# Autodesk Inventor assembly: Dribbler
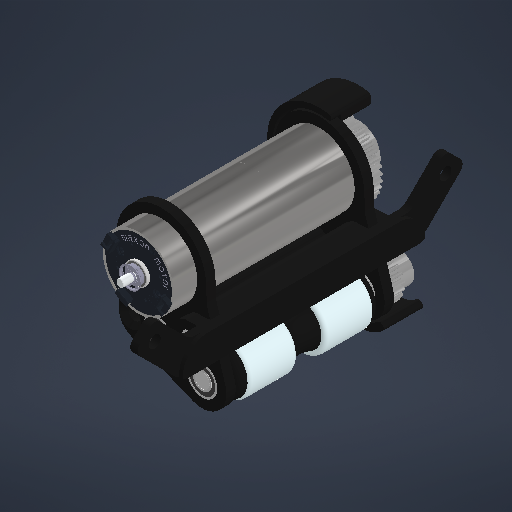
[picture p0: Inventor's stored thumbnail of the model, 512x512]
Saved by Autodesk Inventor 2026.1 (Build 301233020, 233B)
## iProperties
Created: 2025-12-15
Part Number: Dribbler
Document SubType Name: Assembly
Designer: Bahaa
Author: Bahaa
## Documents named in this file (16)
- C:\Users\Bahaa\Nextcloud2\CAD\25-26\Dribbler\Dribbler.iam
- C:\Users\Bahaa\Nextcloud2\CAD\25-26\Dribbler\Dribbler Bracket.ipt
- C:\Users\Bahaa\Nextcloud2\CAD\25-26\Parts\Miniatur Kugellager MR 84 2RS 4x8x3 mm.ipt
- C:\Users\Bahaa\Nextcloud2\CAD\25-26\Motoren\Maxon DCX 19mm 13W\DCX 19mm 13W.iam
- C:\Users\Bahaa\Nextcloud2\CAD\25-26\Dribbler\21102000.ipt
- C:\Users\Bahaa\Nextcloud2\CAD\25-26\Dribbler\21103000.ipt
- C:\Users\Bahaa\Nextcloud2\CAD\25-26\Dribbler\21104000.ipt
- C:\Users\Bahaa\Nextcloud2\CAD\25-26\Dribbler\Dribbler Bracket B.ipt
- C:\Users\Bahaa\Nextcloud2\CAD\25-26\Dribbler\M4 Dribbler Shaft.ipt
- C:\Users\Bahaa\Nextcloud2\CAD\25-26\Dribbler\Dribbler Roller.ipt
- C:\Users\Bahaa\Nextcloud2\CAD\25-26\Dribbler\Dribbler Roller Seperator.ipt
- C:\Users\Bahaa\Nextcloud2\CAD\25-26\Dribbler\Dribbler Support.ipt
- C:\Users\Bahaa\Nextcloud2\CAD\25-26\Dribbler\Dribbler Cover.ipt
- C:\Users\Bahaa\Nextcloud2\CAD\25-26\Dribbler\Dribber Shaft Hull.ipt
- C:\Users\Bahaa\Nextcloud2\CAD\25-26\Dribbler\Dribbler Mount.ipt
- C:\Users\Bahaa\Nextcloud2\CAD\25-26\Dribbler\Pivot M3 Shaft.ipt
## Components (20 placed, 15 different names)
1. Dribbler Bracket:1 — Mate:1, Mate:2, Flush:1, Flush:2, Mate:3, Mate:4, Mate:5, Mate:6, Mate:8, Mate:10, Mate:15, Mate:26, Mate:27, Mate:31, Mate:34, Transitional:1
2. Miniatur Kugellager MR 84 2RS 4x8x3 mm:1 — Mate:1, Flush:2, Mate:9
3. Miniatur Kugellager MR 84 2RS 4x8x3 mm:2 — Mate:2, Flush:1, Mate:11, Mate:36
4. DCX 19mm 13W:1 [sub-assembly] — Mate:3, Mate:4, Mate:5, Mate:7, Mate:12, Flush:5
5. 21102000:1 — Mate:10, Mate:11, Mate:17, Flush:7
6. 21103000:1 — Mate:8, Mate:9, Mate:16, Flush:6
7. 21104000:1 — Mate:6, Mate:7
8. Dribbler Bracket B:1 — Mate:12, Flush:3, Mate:13, Flush:4, Mate:14, Mate:15, Flush:5, Mate:24, Mate:25, Mate:30
9. Miniatur Kugellager MR 84 2RS 4x8x3 mm:3 — Flush:3, Mate:13
10. Miniatur Kugellager MR 84 2RS 4x8x3 mm:4 — Flush:4, Mate:14
11. M4 Dribbler Shaft:1 — Mate:16, Flush:6, Mate:29
12. M4 Dribbler Shaft:2 — Mate:17, Flush:7, Mate:19, Mate:21, Mate:23
13. Dribbler Roller:1 — Mate:19, Mate:38
14. Dribbler Roller:2 — Mate:21, Mate:37
15. Dribbler Roller Seperator:1 — Mate:23, Mate:36, Mate:37, Mate:38
16. Dribbler Support:1 — Mate:24, Mate:25
17. Dribbler Cover:1 — Mate:26, Mate:27, Mate:31
18. Dribber Shaft Hull:1 — Mate:29, Mate:30
19. Dribbler Mount:1 — Mate:32, Mate:33, Flush:8, Mate:34, Mate:35, Flush:9
20. Pivot M3 Shaft:1 — Mate:35, Flush:9, Transitional:1
## Relationships (44: Mate 34, Flush 9, Transitional 1)
- Mate:1: Dribbler Bracket:1 ↔ Miniatur Kugellager MR 84 2RS 4x8x3 mm:1
- Mate:2: Dribbler Bracket:1 ↔ Miniatur Kugellager MR 84 2RS 4x8x3 mm:2
- Flush:1: Dribbler Bracket:1 ↔ Miniatur Kugellager MR 84 2RS 4x8x3 mm:2
- Flush:2: Dribbler Bracket:1 ↔ Miniatur Kugellager MR 84 2RS 4x8x3 mm:1
- Mate:3: Dribbler Bracket:1 ↔ DCX 19mm 13W:1
- Mate:4: Dribbler Bracket:1 ↔ DCX 19mm 13W:1
- Mate:5: Dribbler Bracket:1 ↔ DCX 19mm 13W:1
- Mate:6: Dribbler Bracket:1 ↔ 21104000:1
- Mate:7: DCX 19mm 13W:1 ↔ 21104000:1
- Mate:8: Dribbler Bracket:1 ↔ 21103000:1
- Mate:9: Miniatur Kugellager MR 84 2RS 4x8x3 mm:1 ↔ 21103000:1
- Mate:10: Dribbler Bracket:1 ↔ 21102000:1
- Mate:11: Miniatur Kugellager MR 84 2RS 4x8x3 mm:2 ↔ 21102000:1
- Mate:12: DCX 19mm 13W:1 ↔ Dribbler Bracket B:1
- Flush:3: Dribbler Bracket B:1 ↔ Miniatur Kugellager MR 84 2RS 4x8x3 mm:3
- Mate:13: Dribbler Bracket B:1 ↔ Miniatur Kugellager MR 84 2RS 4x8x3 mm:3
- Flush:4: Dribbler Bracket B:1 ↔ Miniatur Kugellager MR 84 2RS 4x8x3 mm:4
- Mate:14: Dribbler Bracket B:1 ↔ Miniatur Kugellager MR 84 2RS 4x8x3 mm:4
- Mate:15: Dribbler Bracket:1 ↔ Dribbler Bracket B:1
- Flush:5 (-6 mm): DCX 19mm 13W:1 ↔ Dribbler Bracket B:1
- Mate:16: 21103000:1 ↔ M4 Dribbler Shaft:1
- Flush:6: 21103000:1 ↔ M4 Dribbler Shaft:1
- Mate:17: 21102000:1 ↔ M4 Dribbler Shaft:2
- Flush:7: 21102000:1 ↔ M4 Dribbler Shaft:2
- Mate:19: M4 Dribbler Shaft:2 ↔ Dribbler Roller:1
- Mate:21: M4 Dribbler Shaft:2 ↔ Dribbler Roller:2
- Mate:23: M4 Dribbler Shaft:2 ↔ Dribbler Roller Seperator:1
- Mate:24: Dribbler Bracket B:1 ↔ Dribbler Support:1
- Mate:25: Dribbler Bracket B:1 ↔ Dribbler Support:1
- Mate:26: Dribbler Bracket:1 ↔ Dribbler Cover:1
- Mate:27: Dribbler Bracket:1 ↔ Dribbler Cover:1
- Mate:29: M4 Dribbler Shaft:1 ↔ Dribber Shaft Hull:1
- Mate:30: Dribbler Bracket B:1 ↔ Dribber Shaft Hull:1
- Mate:31: Dribbler Bracket:1 ↔ Dribbler Cover:1
- Mate:32: Dribbler Mount:1
- Mate:33: Dribbler Mount:1
- Flush:8: Dribbler Mount:1
- Mate:34 (0.15 mm): Dribbler Bracket:1 ↔ Dribbler Mount:1
- Mate:35: Dribbler Mount:1 ↔ Pivot M3 Shaft:1
- Flush:9: Dribbler Mount:1 ↔ Pivot M3 Shaft:1
- Transitional:1: Dribbler Bracket:1 ↔ Pivot M3 Shaft:1
- Mate:36: Miniatur Kugellager MR 84 2RS 4x8x3 mm:2 ↔ Dribbler Roller Seperator:1
- Mate:37: Dribbler Roller:2 ↔ Dribbler Roller Seperator:1
- Mate:38: Dribbler Roller:1 ↔ Dribbler Roller Seperator:1
